# Autodesk Inventor assembly: Middle Hang Assembly
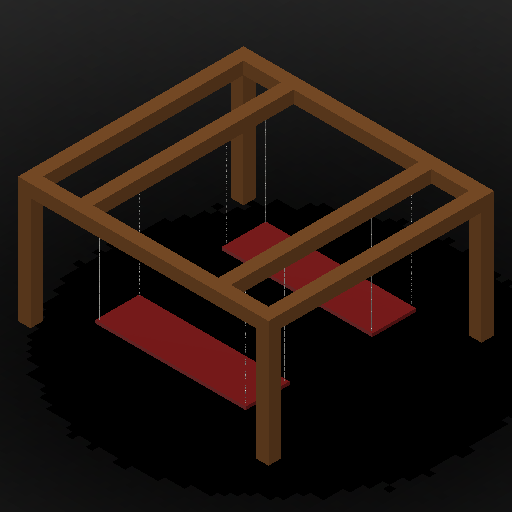
[picture p0: Inventor's stored thumbnail of the model, 512x512]
Saved by Autodesk Inventor 2021 (Build 250183000, 183)
## iProperties
Created: 2021-02-06
Part Number: Middle Hang Assembly
Document SubType Name: Assembly
Designer: aidan
Author: aidan
## Documents named in this file (4)
- C:\Users\Merkileg\Documents\t3-cad\CAD\Game Design\Middle Hang Assembly.iam
- C:\Users\Merkileg\Documents\t3-cad\CAD\Game Design\Hanging Platform.ipt
- C:\Users\Merkileg\Documents\t3-cad\CAD\Game Design\8ft chain.ipt
- C:\Users\Merkileg\Documents\t3-cad\CAD\Game Design\Game Design Truss.ipt
## Components (11 placed, 3 different names)
1. Hanging Platform:1 — Mate:5, Mate:6, Mate:7, Mate:8, Mate:9, Mate:10, Mate:11, Mate:12, Angle:1, Flush:1, Flush:2
2. Hanging Platform:2 — Mate:1, Mate:2, Mate:3, Mate:4, Mate:13, Mate:14, Mate:15, Mate:16, Angle:1, Flush:1, Flush:2, Mate:17, Angle:2, Flush:3
3. 8ft chain:1 — Mate:3, Mate:14
4. 8ft chain:2 — Mate:1, Mate:15
5. 8ft chain:3 — Mate:4, Mate:13
6. 8ft chain:4 — Mate:2, Mate:16
7. 8ft chain:5 — Mate:7, Mate:10
8. 8ft chain:6 — Mate:8, Mate:9
9. 8ft chain:7 — Mate:6, Mate:12
10. 8ft chain:8 — Mate:5, Mate:11
11. Game Design Truss:1 — Mate:17, Angle:2, Flush:3
## Relationships (22: Mate 17, Flush 3, Angle 2)
- Mate:1: Hanging Platform:2 ↔ 8ft chain:2
- Mate:2: Hanging Platform:2 ↔ 8ft chain:4
- Mate:3: Hanging Platform:2 ↔ 8ft chain:1
- Mate:4: Hanging Platform:2 ↔ 8ft chain:3
- Mate:5: Hanging Platform:1 ↔ 8ft chain:8
- Mate:6: Hanging Platform:1 ↔ 8ft chain:7
- Mate:7: Hanging Platform:1 ↔ 8ft chain:5
- Mate:8: Hanging Platform:1 ↔ 8ft chain:6
- Mate:9: Hanging Platform:1 ↔ 8ft chain:6
- Mate:10: Hanging Platform:1 ↔ 8ft chain:5
- Mate:11: Hanging Platform:1 ↔ 8ft chain:8
- Mate:12: Hanging Platform:1 ↔ 8ft chain:7
- Mate:13: Hanging Platform:2 ↔ 8ft chain:3
- Mate:14: Hanging Platform:2 ↔ 8ft chain:1
- Mate:15: Hanging Platform:2 ↔ 8ft chain:2
- Mate:16: Hanging Platform:2 ↔ 8ft chain:4
- Angle:1 (0 deg): Hanging Platform:1 ↔ Hanging Platform:2
- Flush:1: Hanging Platform:1 ↔ Hanging Platform:2
- Flush:2: Hanging Platform:1 ↔ Hanging Platform:2
- Mate:17 (2438.4 mm): Hanging Platform:2 ↔ Game Design Truss:1
- Angle:2 (90 deg): Hanging Platform:2 ↔ Game Design Truss:1
- Flush:3: Hanging Platform:2 ↔ Game Design Truss:1
